# Autodesk Inventor assembly: school desk
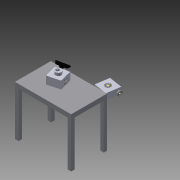
[picture p0: Inventor's stored thumbnail of the model, 180x180]
Saved by Autodesk Inventor 2015 (Build 190159000, 159)
## iProperties
Created: 2014-10-26
Part Number: school desk
Document SubType Name: Assembly
Designer: ericd_000
Author: ericd_000
## Documents named in this file (8)
- C:\Users\ericd_000\Dropbox\GitHub\initial_cad\eric_cad\school desk.iam
- C:\Users\ericd_000\Dropbox\GitHub\initial_cad\eric_cad\tables.ipt
- C:\Users\ericd_000\Dropbox\GitHub\initial_cad\eric_cad\bottom box with container\bottom box with container-01.iam
- C:\Users\ericd_000\Dropbox\GitHub\initial_cad\eric_cad\bottom box with container.iam
- C:\Users\ericd_000\Dropbox\GitHub\initial_cad\eric_cad\perception module\perception module-01.iam
- C:\Users\ericd_000\Dropbox\GitHub\initial_cad\eric_cad\perception module.iam
- C:\Users\ericd_000\Dropbox\GitHub\initial_cad\eric_cad\locomotion assembly\locomotion assembly-01.iam
- C:\Users\ericd_000\Dropbox\GitHub\initial_cad\eric_cad\locomotion assembly.iam
## Components (4 placed, 4 different names)
1. tables:1 — Mate:2, Flush:1
2. bottom box with container-01:1 [sub-assembly] — Mate:1, Mate:2, Mate:3
3. perception module-01:1 [sub-assembly] — Mate:1, Mate:3
4. locomotion assembly-01:1 [sub-assembly] — Flush:1
## Relationships (4: Mate 3, Flush 1)
- Mate:1: bottom box with container-01:1 ↔ perception module-01:1
- Mate:2: tables:1 ↔ bottom box with container-01:1
- Mate:3: bottom box with container-01:1 ↔ perception module-01:1
- Flush:1 (10 mm): tables:1 ↔ locomotion assembly-01:1
